# Autodesk Inventor assembly: s-assy-shooter_frame_light
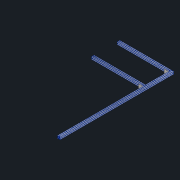
[picture p0: Inventor's stored thumbnail of the model, 180x180]
Saved by Autodesk Inventor 2022 (Build 260153000, 153)
## iProperties
Created: 2021-09-11
Part Number: s-assy-shooter_frame_light
Document SubType Name: Assembly
Designer: yuto6
Mass: 2250.1 g
Surface Area: 6706.14 cm^2
Volume: 745.503 cm^3
Density: 3.01823 g/cm^3
Author: yuto6
## Documents named in this file (5)
- C:\Users\yuta0\Documents\GitHub\catchrobo_hardware\assy-shooter\s-assy-shooter_frame_light.iam
- C:\Users\yuta0\Documents\GitHub\catchrobo_hardware\assy-shooter\s-assy-blacket.iam
- C:\Users\yuta0\Documents\GitHub\catchrobo_hardware\assy-shooter\HNTC5-5.iam
- C:\Users\yuta0\Documents\GitHub\catchrobo_hardware\assy-shooter\NFS5-2020-351.ipt
- C:\Users\yuta0\Documents\GitHub\catchrobo_hardware\assy-shooter\NFS5-2020-885.ipt
## Components (9 placed, 4 different names)
1. NFS5-2020-885:1 — メイト:4, フラッシュ:5, フラッシュ:6, メイト:12, フラッシュ:10
2. s-assy-blacket:5 [sub-assembly] — メイト:11, メイト:12, フラッシュ:10
3. NFS5-2020-351:1 — メイト:4, フラッシュ:5, フラッシュ:6, メイト:11, メイト:13, メイト:14, メイト:21, メイト:22
4. HNTC5-5:3 [sub-assembly] — メイト:21, メイト:22, メイト:24
5. HNTC5-5:1 [sub-assembly] — メイト:13, メイト:14, メイト:24
6. s-assy-blacket:6 [sub-assembly]
7. NFS5-2020-351:2
8. HNTC5-5:4 [sub-assembly]
9. HNTC5-5:5 [sub-assembly]
## Component patterns: (2 elements, first: s-assy-blacket:5 + NFS5-2020-351:1 + HNTC5-5:3 + HNTC5-5:1)
## Relationships (11: Mate 8, Flush 3)
- メイト:4 [Mate]: NFS5-2020-885:1 ↔ NFS5-2020-351:1
- フラッシュ:5 [Flush]: NFS5-2020-885:1 ↔ NFS5-2020-351:1
- フラッシュ:6 [Flush]: NFS5-2020-885:1 ↔ NFS5-2020-351:1
- メイト:11 [Mate]: s-assy-blacket:5 ↔ NFS5-2020-351:1
- メイト:12 [Mate]: NFS5-2020-885:1 ↔ s-assy-blacket:5
- フラッシュ:10 [Flush]: NFS5-2020-885:1 ↔ s-assy-blacket:5
- メイト:13 [Mate]: NFS5-2020-351:1 ↔ HNTC5-5:1
- メイト:14 [Mate] (0.1 mm): NFS5-2020-351:1 ↔ HNTC5-5:1
- メイト:21 [Mate] (0.1 mm): NFS5-2020-351:1 ↔ HNTC5-5:3
- メイト:22 [Mate]: NFS5-2020-351:1 ↔ HNTC5-5:3
- メイト:24 [Mate] (160 mm): HNTC5-5:3 ↔ HNTC5-5:1
